# Autodesk Inventor assembly: SM_XA01
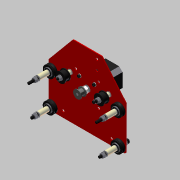
[picture p0: Inventor's stored thumbnail of the model, 180x180]
Saved by Autodesk Inventor 2012 SP1 (Build 160190100, 190)
## iProperties
Created: 2012-05-01
Part Number: SM_XA01
Document SubType Name: Assembly
Designer: ERF
Description: X Axis Motor Mount Plate
Stock Number: SM_XA01
Author: ERF
Title: X Axis Motor Mount Plate Assembly
## Documents named in this file (15)
- C:\Users\eford\Documents\Projects\Shapoko_v1i\Workspaces\Workspace\Projects\USER FOLDER\Edward\Shapeoko_v1i\Assemblies\SM-XA01.iam
- C:\Users\eford\Documents\Projects\Shapoko_v1i\Workspaces\Workspace\Projects\USER FOLDER\Edward\Shapeoko_v1i\Parts\SM-H04.ipt
- C:\Users\eford\Documents\Projects\Shapoko_v1i\Workspaces\Workspace\Projects\USER FOLDER\Edward\Shapeoko_v1i\Parts\SM-H01.ipt
- C:\Users\eford\Documents\Projects\Shapoko_v1i\Workspaces\Workspace\Projects\USER FOLDER\Edward\Shapeoko_v1i\Parts\MSK01-04.ipt
- C:\Users\eford\Documents\Projects\Shapoko_v1i\Workspaces\Workspace\Projects\USER FOLDER\Edward\Shapeoko_v1i\Parts\SM-H08.ipt
- C:\Users\eford\Documents\Projects\Shapoko_v1i\Workspaces\Workspace\Projects\USER FOLDER\Edward\Shapeoko_v1i\Parts\SM-S01.ipt
- C:\Users\eford\Documents\Projects\Shapoko_v1i\Workspaces\Workspace\Projects\USER FOLDER\Edward\Shapeoko_v1i\Parts\MSK01-09.ipt
- C:\Users\eford\Documents\Projects\Shapoko_v1i\Workspaces\Workspace\Projects\USER FOLDER\Edward\Shapeoko_v1i\Parts\SM-E01.ipt
- C:\Users\eford\Documents\Projects\Shapoko_v1i\Workspaces\Workspace\Projects\USER FOLDER\Edward\Shapeoko_v1i\Parts\SM-H03.ipt
- C:\Users\eford\Documents\Projects\Shapoko_v1i\Workspaces\Workspace\Projects\USER FOLDER\Edward\Shapeoko_v1i\Parts\SM-H14.ipt
- C:\Users\eford\Documents\Projects\Shapoko_v1i\Workspaces\Workspace\Projects\USER FOLDER\Edward\Shapeoko_v1i\Parts\SM-H15.ipt
- C:\Users\eford\Documents\Projects\Shapoko_v1i\Workspaces\Workspace\Projects\USER FOLDER\Edward\Shapeoko_v1i\Parts\SM-H09.ipt
- C:\Users\eford\Documents\Projects\Shapoko_v1i\Workspaces\Workspace\Projects\USER FOLDER\Edward\Shapeoko_v1i\Parts\SM-H02.ipt
- C:\Users\eford\Documents\Projects\Shapoko_v1i\Workspaces\Workspace\Projects\USER FOLDER\Edward\Shapeoko_v1i\Assemblies\MSK01-06A.iam
- C:\Users\eford\Documents\Projects\Shapoko_v1i\Workspaces\Workspace\Projects\USER FOLDER\Edward\Shapeoko_v1i\Assemblies\MSK01-05A.iam
## Components (65 placed, 14 different names)
1. SM-H04:1 — Insert:55
2. SM-H01:1 — Insert:26, Insert:28
3. SM-H04:2 — Insert:54
4. SM-H04:3 — Insert:53
5. MSK01-04:1 — Insert:5, Insert:8
6. SM-H04:4 — Insert:52
7. SM-H01:2 — Insert:25, Insert:27
8. SM-H04:5 — Insert:51
9. MSK01-04:2 — Insert:6, Insert:7
10. SM-H04:6 — Insert:50
11. SM-H08:1 — Insert:9
12. SM-H08:2 — Insert:10
13. SM-S01:1 — Insert:7, Insert:8, Insert:11, Insert:12, Insert:13, Insert:14, Insert:16, Insert:17, Insert:37, Mate:4, Mate:5, Mate:6, Insert:56, Angle:1, Insert:61, Insert:62, Insert:63, Insert:64
14. MSK01-06A:3 [sub-assembly] — Insert:66, Insert:67
15. MSK01-06A:4 [sub-assembly] — Insert:68, Insert:69
16. MSK01-09:1 — Insert:65
17. MSK01-05A:5 [sub-assembly] — Insert:70, Insert:71
18. MSK01-05A:6 [sub-assembly] — Insert:76, Insert:77
19. MSK01-05A:7 [sub-assembly] — Insert:74, Insert:75
20. MSK01-05A:8 [sub-assembly] — Insert:72, Insert:73
21. SM-E01:1 — Insert:56, Angle:1, Insert:65
22. SM-H09:2 — Insert:1, Mate:3, Mate:8
23. SM-H09:3 — Insert:4, Mate:1, Mate:10
24. SM-H09:4 — Insert:2
25. SM-H09:5 — Insert:3, Mate:7
26. SM-H03:2 — Insert:1, Insert:5
27. SM-H03:3 — Insert:2, Insert:13
28. SM-H03:4 — Insert:3, Insert:14
29. SM-H03:5 — Insert:4, Insert:6
30. SM-H03:6 — Insert:10, Insert:12
31. SM-H03:7 — Insert:9, Insert:11
32. SM-H03:8 — Insert:22, Insert:76
33. SM-H03:9 — Insert:21, Insert:70
34. SM-H03:10 — Insert:16, Insert:25
35. SM-H03:11 — Insert:17, Insert:26
36. SM-H03:12 — Insert:24, Insert:74
37. SM-H03:13 — Insert:23, Insert:72
38. SM-H02:2 — Insert:21, Insert:33
39. SM-H02:3 — Insert:23, Insert:36
40. SM-H02:4 — Insert:22, Insert:34
41. SM-H02:5 — Insert:24, Insert:35
42. SM-H03:14 — Insert:27, Insert:68
43. SM-H03:15 — Insert:28, Insert:66
44. SM-H03:16 — Insert:55, Insert:67
45. SM-H03:17 — Insert:54, Insert:69
46. SM-H03:18 — Insert:36
47. SM-H03:19 — Insert:35
48. SM-H03:20 — Insert:33
49. SM-H03:21 — Insert:34
50. SM-H03:22 — Mate:3, Mate:5, Insert:75
51. SM-H03:23 — Mate:6, Mate:7, Insert:73
52. SM-H03:25 — Mate:1, Mate:4, Insert:77
53. SM-H03:26 — Insert:37, Insert:71
54. SM-H03:27 — Insert:52
55. SM-H03:28 — Mate:8, Insert:53
56. SM-H03:29 — Insert:51
57. SM-H03:30 — Mate:10, Insert:50
58. SM-H15:2 — Insert:57, Insert:64
59. SM-H14:2 — Insert:57
60. SM-H15:3 — Insert:58, Insert:62
61. SM-H14:3 — Insert:58
62. SM-H15:4 — Insert:60, Insert:63
63. SM-H14:4 — Insert:60
64. SM-H15:5 — Insert:59, Insert:61
65. SM-H14:5 — Insert:59
## Relationships (66: Insert 57, Mate 8, Angle 1)
- Insert:1: SM-H09:2 ↔ SM-H03:2
- Insert:2: SM-H09:4 ↔ SM-H03:3
- Insert:3: SM-H09:5 ↔ SM-H03:4
- Insert:4: SM-H09:3 ↔ SM-H03:5
- Insert:5: MSK01-04:1 ↔ SM-H03:2
- Insert:6: MSK01-04:2 ↔ SM-H03:5
- Insert:7: MSK01-04:2 ↔ SM-S01:1
- Insert:8: MSK01-04:1 ↔ SM-S01:1
- Insert:9: SM-H08:1 ↔ SM-H03:7
- Insert:10: SM-H08:2 ↔ SM-H03:6
- Insert:11: SM-S01:1 ↔ SM-H03:7
- Insert:12: SM-S01:1 ↔ SM-H03:6
- Insert:13: SM-S01:1 ↔ SM-H03:3
- Insert:14: SM-S01:1 ↔ SM-H03:4
- Insert:16: SM-S01:1 ↔ SM-H03:10
- Insert:17: SM-S01:1 ↔ SM-H03:11
- Insert:21: SM-H03:9 ↔ SM-H02:2
- Insert:22: SM-H03:8 ↔ SM-H02:4
- Insert:23: SM-H03:13 ↔ SM-H02:3
- Insert:24: SM-H03:12 ↔ SM-H02:5
- Insert:25: SM-H01:2 ↔ SM-H03:10
- Insert:26: SM-H01:1 ↔ SM-H03:11
- Insert:27: SM-H01:2 ↔ SM-H03:14
- Insert:28: SM-H01:1 ↔ SM-H03:15
- Insert:33: SM-H02:2 ↔ SM-H03:20
- Insert:34: SM-H02:4 ↔ SM-H03:21
- Insert:35: SM-H02:5 ↔ SM-H03:19
- Insert:36: SM-H02:3 ↔ SM-H03:18
- Mate:1: SM-H09:3 ↔ SM-H03:25
- Mate:3: SM-H09:2 ↔ SM-H03:22
- Insert:37: SM-S01:1 ↔ SM-H03:26
- Mate:4: SM-S01:1 ↔ SM-H03:25
- Mate:5: SM-S01:1 ↔ SM-H03:22
- Mate:6: SM-S01:1 ↔ SM-H03:23
- Mate:7: SM-H09:5 ↔ SM-H03:23
- Mate:8: SM-H09:2 ↔ SM-H03:28
- Mate:10: SM-H09:3 ↔ SM-H03:30
- Insert:50: SM-H04:6 ↔ SM-H03:30
- Insert:51: SM-H04:5 ↔ SM-H03:29
- Insert:52: SM-H04:4 ↔ SM-H03:27
- Insert:53: SM-H04:3 ↔ SM-H03:28
- Insert:54: SM-H04:2 ↔ SM-H03:17
- Insert:55: SM-H04:1 ↔ SM-H03:16
- Insert:56: SM-S01:1 ↔ SM-E01:1
- Angle:1 (0 deg): SM-S01:1 ↔ SM-E01:1
- Insert:57: SM-H15:2 ↔ SM-H14:2
- Insert:58: SM-H15:3 ↔ SM-H14:3
- Insert:59: SM-H15:5 ↔ SM-H14:5
- Insert:60: SM-H15:4 ↔ SM-H14:4
- Insert:61: SM-S01:1 ↔ SM-H15:5
- Insert:62: SM-S01:1 ↔ SM-H15:3
- Insert:63: SM-S01:1 ↔ SM-H15:4
- Insert:64: SM-S01:1 ↔ SM-H15:2
- Insert:65 (5.08 mm): MSK01-09:1 ↔ SM-E01:1
- Insert:66: MSK01-06A:3 ↔ SM-H03:15
- Insert:67: MSK01-06A:3 ↔ SM-H03:16
- Insert:68: MSK01-06A:4 ↔ SM-H03:14
- Insert:69: MSK01-06A:4 ↔ SM-H03:17
- Insert:70: MSK01-05A:5 ↔ SM-H03:9
- Insert:71: MSK01-05A:5 ↔ SM-H03:26
- Insert:72: MSK01-05A:8 ↔ SM-H03:13
- Insert:73: MSK01-05A:8 ↔ SM-H03:23
- Insert:74: MSK01-05A:7 ↔ SM-H03:12
- Insert:75: MSK01-05A:7 ↔ SM-H03:22
- Insert:76: MSK01-05A:6 ↔ SM-H03:8
- Insert:77: MSK01-05A:6 ↔ SM-H03:25
